# Autodesk Inventor assembly: Rear_Frame_Fixer
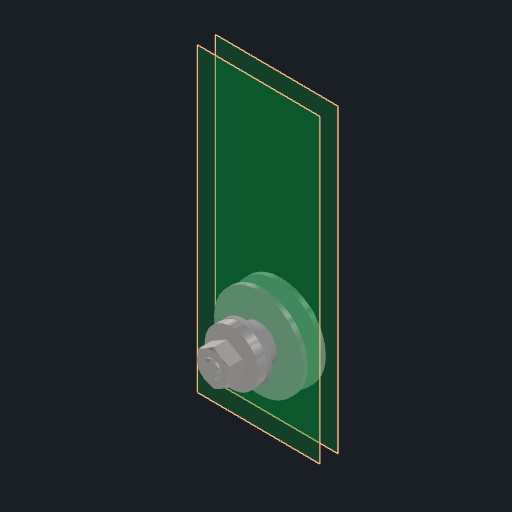
[picture p0: Inventor's stored thumbnail of the model, 512x512]
Saved by Autodesk Inventor 2024.3 (Build 283343000, 343)
## iProperties
Created: 2024-01-28
Part Number: Rear_Frame_Fixer
Document SubType Name: Assembly
Designer: 김대겸
Author: 김대겸
## Documents named in this file (7)
- C:\Users\ASUS\Desktop\test\v2_Frame\Rear_Frame_Fixer.iam
- C:\Users\ASUS\Desktop\test\v1_Frame\MISUMI\C-WSSA12-4-2.ipt
- C:\Users\ASUS\Desktop\test\v1_Frame\MISUMI\80F-0606.ipt
- C:\Users\ASUS\Desktop\test\v2_Frame\Handmade tiered cover_9mm.ipt
- C:\Users\ASUS\Desktop\test\v1_Frame\MISUMI\SLBNR4.ipt
- C:\Users\ASUS\Desktop\test\v2_Frame\MISUMI\CSHBTT-ST-M4-18.ipt
- C:\Users\ASUS\Desktop\test\v2_Frame\MISUMI\WSSS20-8-1.ipt
## Components (7 placed, 6 different names)
1. C-WSSA12-4-2:1 — 삽입:1, 삽입:2
2. 80F-0606:1 — 삽입:2, 삽입:5, 삽입:7
3. Handmade tiered cover_9mm:1 — 삽입:5, 삽입:6
4. SLBNR4:1 — 삽입:1
5. CSHBTT-ST-M4-18:1 — 삽입:6
6. WSSS20-8-1:1 — 삽입:7, 삽입:8
7. WSSS20-8-1:2 — 삽입:8
## Relationships (6: Insert 6)
- 삽입:1 [Insert] (1 mm): C-WSSA12-4-2:1 ↔ SLBNR4:1
- 삽입:2 [Insert]: C-WSSA12-4-2:1 ↔ 80F-0606:1
- 삽입:5 [Insert]: 80F-0606:1 ↔ Handmade tiered cover_9mm:1
- 삽입:6 [Insert]: Handmade tiered cover_9mm:1 ↔ CSHBTT-ST-M4-18:1
- 삽입:7 [Insert] (3 mm): 80F-0606:1 ↔ WSSS20-8-1:1
- 삽입:8 [Insert] (3 mm): WSSS20-8-1:1 ↔ WSSS20-8-1:2
